# Autodesk Inventor assembly: Car assembly
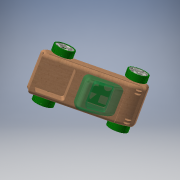
[picture p0: Inventor's stored thumbnail of the model, 180x180]
Saved by Autodesk Inventor 2017 (Build 210142000, 142)
## iProperties
Created: 2017-03-23
Part Number: Car assembly
Document SubType Name: Assembly
Designer: 196918
Author: 196918
## Documents named in this file (12)
- C:\Users\rbibb\Desktop\Car assembly.iam
- C:\Users\rbibb\Desktop\T9 Axle (1).ipt
- C:\Users\rbibb\Desktop\T9 Bed.ipt
- C:\Users\rbibb\Desktop\T9 Connector.ipt
- C:\Users\rbibb\Desktop\T9 Front.ipt
- C:\Users\rbibb\Desktop\T9 One Block Socket.ipt
- C:\Users\rbibb\Desktop\T9 Passenger Base.ipt
- C:\Users\rbibb\Desktop\T9 Passenger Section.ipt
- C:\Users\rbibb\Desktop\T9 Tire.ipt
- C:\Users\rbibb\Desktop\T9 Two Block Socket.ipt
- C:\Users\rbibb\Desktop\T9 Wheel (1).ipt
- C:\Users\rbibb\Desktop\T9 Windshield.ipt
## Components (23 placed, 11 different names)
1. T9 Connector:1 — Mate:6, Rigid:2
2. T9 Front:1 — Rotational:3, Rotational:4, Rigid:3, Mate:11, Flush:1, Mate:12
3. T9 One Block Socket:1 — Rigid:1, Mate:6
4. T9 Passenger Base:1 — Mate:1, Mate:2, Mate:7, Mate:8
5. T9 Passenger Section:1 — Mate:1, Mate:2, Rigid:1, Mate:7, Mate:8, Mate:9, Rigid:5, Mate:11, Flush:1, Mate:12, Mate:13, Mate:14, Mate:15, Flush:2, Flush:3
6. T9 Two Block Socket:1 — Rigid:2, Rigid:3
7. T9 Windshield:1 — Mate:9, Mate:13, Mate:14, Mate:15
8. T9 Axle (1):3 — Rotational:4, Rigid:4
9. T9 Axle (1):4 — Rotational:3, Rotational:8
10. T9 Tire:2
11. T9 Wheel (1):2 — Rotational:8
12. T9 Tire:4
13. T9 Wheel (1):4 — Rigid:4
14. T9 One Block Socket:2 — Rigid:7, Mate:16
15. T9 Two Block Socket:2 — Rigid:5, Rigid:6
16. T9 Connector:2 — Rigid:6, Rigid:7
17. T9 Bed:1 — Mate:16, Flush:2, Flush:3, Rotational:10, Rotational:12
18. T9 Axle (1):5 — Rotational:10, Rotational:11
19. T9 Axle (1):6 — Rotational:12, Rotational:13
20. T9 Wheel (1):5 — Rotational:13, Rotational:14
21. T9 Wheel (1):6 — Rotational:11, Rotational:15
22. T9 Tire:5 — Rotational:14
23. T9 Tire:6 — Rotational:15
## Relationships (33: Mate 12, RevoluteJoint 11, WeldJoint 7, Flush 3)
- Mate:1: T9 Passenger Base:1 ↔ T9 Passenger Section:1
- Mate:2: T9 Passenger Base:1 ↔ T9 Passenger Section:1
- Rigid:1 [WeldJoint]: T9 One Block Socket:1 ↔ T9 Passenger Section:1
- Mate:6: T9 Connector:1 ↔ T9 One Block Socket:1
- Rotational:3 [RevoluteJoint]: T9 Front:1 ↔ T9 Axle (1):4
- Rotational:4 [RevoluteJoint]: T9 Front:1 ↔ T9 Axle (1):3
- Mate:7: T9 Passenger Base:1 ↔ T9 Passenger Section:1
- Mate:8: T9 Passenger Base:1 ↔ T9 Passenger Section:1
- Mate:9: T9 Passenger Section:1 ↔ T9 Windshield:1
- Rigid:2 [WeldJoint]: T9 Connector:1 ↔ T9 Two Block Socket:1
- Rigid:3 [WeldJoint]: T9 Front:1 ↔ T9 Two Block Socket:1
- [RevoluteJoint]: T9 Tire:2 ↔ T9 Wheel (1):2
- [RevoluteJoint]: T9 Tire:4 ↔ T9 Wheel (1):4
- Rigid:4 [WeldJoint]: T9 Axle (1):3 ↔ T9 Wheel (1):4
- Rotational:8 [RevoluteJoint]: T9 Axle (1):4 ↔ T9 Wheel (1):2
- Rigid:5 [WeldJoint]: T9 Passenger Section:1 ↔ T9 Two Block Socket:2
- Rigid:6 [WeldJoint]: T9 Two Block Socket:2 ↔ T9 Connector:2
- Rigid:7 [WeldJoint]: T9 One Block Socket:2 ↔ T9 Connector:2
- Mate:11: T9 Front:1 ↔ T9 Passenger Section:1
- Flush:1: T9 Front:1 ↔ T9 Passenger Section:1
- Mate:12 (-58.166 mm): T9 Front:1 ↔ T9 Passenger Section:1
- Mate:13: T9 Passenger Section:1 ↔ T9 Windshield:1
- Mate:14: T9 Passenger Section:1 ↔ T9 Windshield:1
- Mate:15: T9 Passenger Section:1 ↔ T9 Windshield:1
- Mate:16: T9 One Block Socket:2 ↔ T9 Bed:1
- Flush:2: T9 Passenger Section:1 ↔ T9 Bed:1
- Flush:3: T9 Passenger Section:1 ↔ T9 Bed:1
- Rotational:10 [RevoluteJoint]: T9 Bed:1 ↔ T9 Axle (1):5
- Rotational:11 [RevoluteJoint]: T9 Axle (1):5 ↔ T9 Wheel (1):6
- Rotational:12 [RevoluteJoint]: T9 Bed:1 ↔ T9 Axle (1):6
- Rotational:13 [RevoluteJoint]: T9 Axle (1):6 ↔ T9 Wheel (1):5
- Rotational:14 [RevoluteJoint] (13.97 mm): T9 Wheel (1):5 ↔ T9 Tire:5
- Rotational:15 [RevoluteJoint] (13.97 mm): T9 Wheel (1):6 ↔ T9 Tire:6
## Named parameters: d21_d5 = 0 mm, d22_d6 = 45.3338 deg, d25_d5 = 0 mm, d26_d6 = 24.995456 deg
